# Autodesk Inventor assembly: Mounting Part figureing outness
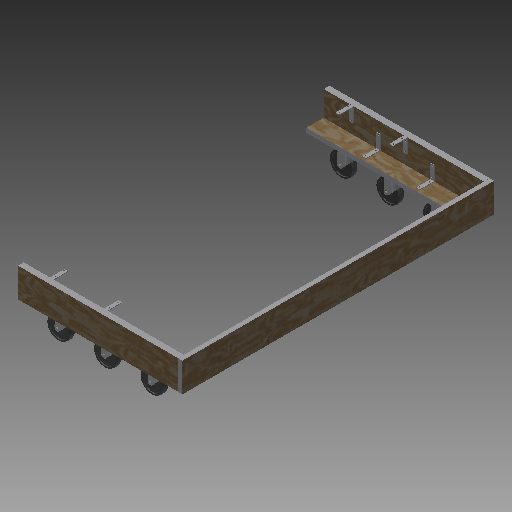
[picture p0: Inventor's stored thumbnail of the model, 512x512]
Saved by Autodesk Inventor 2018.2 (Build 222227000, 227)
## iProperties
Created: 2018-02-21
Part Number: Mounting Part figureing outness
Document SubType Name: Assembly
Designer: owner
Author: owner
## Documents named in this file (7)
- Z:\The Pickle\Final Carts\Mellie Cart\Mounting Part figureing outness.iam
- Z:\The Pickle\Final Carts\WHEELS.ipt
- Z:\The Pickle\Final Carts\Mellie Cart\Wheel mounting side part.ipt
- Z:\The Pickle\Final Carts\Mellie Cart\Wheel mount bottom.ipt
- Z:\The Pickle\Final Carts\Locking Mech\Plywood Pickle Mount Corner Bracket.ipt
- Z:\The Pickle\Final Carts\Locking Mech\Plywood Pickle Mount Triangle Bracket.ipt
- Z:\The Pickle\Final Carts\Mellie Cart\wheel mount front.ipt
## Components (21 placed, 6 different names)
1. Wheel mounting side part:1 — Mate:1, Flush:8, Mate:3, Mate:6, Mate:7, Mate:10, Mate:11, Flush:14, Flush:20, Mate:23, Flush:21
2. Wheel mount bottom:1 — Mate:1, Mate:2, Mate:4, Mate:5, Flush:30, Mate:31
3. WHEELS:1 — Flush:24, Flush:27, Flush:31, Mate:28, Mate:29, Flush:32
4. WHEELS:2 — Flush:23, Flush:28, Flush:34
5. WHEELS:3 — Flush:22, Flush:23, Flush:28, Flush:29, Flush:33
6. WHEELS:4 — Flush:24, Flush:25, Flush:26, Mate:29, Mate:30, Flush:33
7. WHEELS:5 — Flush:25, Flush:26, Flush:27, Mate:27, Mate:30, Flush:34
8. WHEELS:6 — Flush:22, Flush:29, Flush:30, Flush:32, Mate:31
9. Plywood Pickle Mount Corner Bracket:1 — Mate:4, Mate:10, Flush:18, Mate:26
10. Plywood Pickle Mount Triangle Bracket:1 — Flush:8, Mate:2, Mate:3
11. Plywood Pickle Mount Corner Bracket:2 — Mate:6, Flush:17, Mate:25, Mate:26
12. Plywood Pickle Mount Corner Bracket:5 — Mate:18, Mate:20, Flush:18
13. Plywood Pickle Mount Corner Bracket:6 — Mate:17, Flush:13, Flush:17
14. Plywood Pickle Mount Corner Bracket:7 — Mate:16, Mate:19, Flush:16
15. Plywood Pickle Mount Corner Bracket:8 — Mate:15, Flush:12, Flush:15
16. Plywood Pickle Mount Triangle Bracket:8 — Mate:13, Mate:14, Flush:11
17. Plywood Pickle Mount Corner Bracket:9 — Mate:7, Flush:15, Flush:21, Mate:24
18. Plywood Pickle Mount Corner Bracket:10 — Mate:5, Mate:11, Flush:16, Mate:24, Mate:25
19. Wheel mount bottom:2 — Mate:12, Flush:9, Flush:10, Mate:14, Mate:19, Mate:20, Flush:31, Mate:27
20. Wheel mounting side part:2 — Mate:12, Flush:9, Flush:10, Mate:13, Flush:11, Mate:15, Mate:16, Mate:17, Mate:18, Flush:12, Flush:13, Flush:14
21. wheel mount front:1 — Flush:20, Mate:23, Mate:28
## Relationships (53: Mate 27, Flush 26)
- Mate:1: Wheel mounting side part:1 ↔ Wheel mount bottom:1
- Flush:8: Wheel mounting side part:1 ↔ Plywood Pickle Mount Triangle Bracket:1
- Mate:2: Wheel mount bottom:1 ↔ Plywood Pickle Mount Triangle Bracket:1
- Mate:3: Wheel mounting side part:1 ↔ Plywood Pickle Mount Triangle Bracket:1
- Mate:4: Wheel mount bottom:1 ↔ Plywood Pickle Mount Corner Bracket:1
- Mate:5: Wheel mount bottom:1 ↔ Plywood Pickle Mount Corner Bracket:10
- Mate:6: Wheel mounting side part:1 ↔ Plywood Pickle Mount Corner Bracket:2
- Mate:7: Wheel mounting side part:1 ↔ Plywood Pickle Mount Corner Bracket:9
- Mate:10: Wheel mounting side part:1 ↔ Plywood Pickle Mount Corner Bracket:1
- Mate:11: Wheel mounting side part:1 ↔ Plywood Pickle Mount Corner Bracket:10
- Mate:12: Wheel mount bottom:2 ↔ Wheel mounting side part:2
- Flush:9: Wheel mount bottom:2 ↔ Wheel mounting side part:2
- Flush:10: Wheel mount bottom:2 ↔ Wheel mounting side part:2
- Mate:13: Plywood Pickle Mount Triangle Bracket:8 ↔ Wheel mounting side part:2
- Mate:14: Plywood Pickle Mount Triangle Bracket:8 ↔ Wheel mount bottom:2
- Flush:11: Plywood Pickle Mount Triangle Bracket:8 ↔ Wheel mounting side part:2
- Mate:15: Plywood Pickle Mount Corner Bracket:8 ↔ Wheel mounting side part:2
- Mate:16: Plywood Pickle Mount Corner Bracket:7 ↔ Wheel mounting side part:2
- Mate:17: Plywood Pickle Mount Corner Bracket:6 ↔ Wheel mounting side part:2
- Mate:18: Plywood Pickle Mount Corner Bracket:5 ↔ Wheel mounting side part:2
- Flush:12: Plywood Pickle Mount Corner Bracket:8 ↔ Wheel mounting side part:2
- Flush:13: Plywood Pickle Mount Corner Bracket:6 ↔ Wheel mounting side part:2
- Mate:19: Plywood Pickle Mount Corner Bracket:7 ↔ Wheel mount bottom:2
- Mate:20: Plywood Pickle Mount Corner Bracket:5 ↔ Wheel mount bottom:2
- Flush:14: Wheel mounting side part:1 ↔ Wheel mounting side part:2
- Flush:15: Plywood Pickle Mount Corner Bracket:8 ↔ Plywood Pickle Mount Corner Bracket:9
- Flush:16: Plywood Pickle Mount Corner Bracket:7 ↔ Plywood Pickle Mount Corner Bracket:10
- Flush:17: Plywood Pickle Mount Corner Bracket:2 ↔ Plywood Pickle Mount Corner Bracket:6
- Flush:18: Plywood Pickle Mount Corner Bracket:1 ↔ Plywood Pickle Mount Corner Bracket:5
- Flush:20: Wheel mounting side part:1 ↔ wheel mount front:1
- Mate:23: Wheel mounting side part:1 ↔ wheel mount front:1
- Flush:21 (114.3 mm): Wheel mounting side part:1 ↔ Plywood Pickle Mount Corner Bracket:9
- Mate:24 (101.6 mm): Plywood Pickle Mount Corner Bracket:9 ↔ Plywood Pickle Mount Corner Bracket:10
- Mate:25 (101.6 mm): Plywood Pickle Mount Corner Bracket:2 ↔ Plywood Pickle Mount Corner Bracket:10
- Mate:26 (101.6 mm): Plywood Pickle Mount Corner Bracket:1 ↔ Plywood Pickle Mount Corner Bracket:2
- Flush:22: WHEELS:3 ↔ WHEELS:6
- Flush:23: WHEELS:2 ↔ WHEELS:3
- Flush:24: WHEELS:1 ↔ WHEELS:4
- Flush:25: WHEELS:4 ↔ WHEELS:5
- Flush:26: WHEELS:4 ↔ WHEELS:5
- Flush:27: WHEELS:1 ↔ WHEELS:5
- Flush:28: WHEELS:2 ↔ WHEELS:3
- Flush:29: WHEELS:3 ↔ WHEELS:6
- Flush:30 (6.35 mm): Wheel mount bottom:1 ↔ WHEELS:6
- Flush:31 (6.35 mm): WHEELS:1 ↔ Wheel mount bottom:2
- Mate:27: WHEELS:5 ↔ Wheel mount bottom:2
- Mate:28 (107.7976 mm): WHEELS:1 ↔ wheel mount front:1
- Mate:29 (107.7976 mm): WHEELS:1 ↔ WHEELS:4
- Mate:30 (107.7976 mm): WHEELS:4 ↔ WHEELS:5
- Flush:32: WHEELS:1 ↔ WHEELS:6
- Flush:33: WHEELS:3 ↔ WHEELS:4
- Flush:34: WHEELS:2 ↔ WHEELS:5
- Mate:31: Wheel mount bottom:1 ↔ WHEELS:6
